# Autodesk Inventor assembly: Assembly1
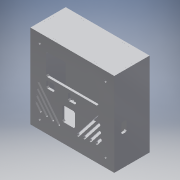
[picture p0: Inventor's stored thumbnail of the model, 180x180]
Saved by Autodesk Inventor 2018.2 (Build 222227000, 227)
## iProperties
Created: 2018-04-05
Part Number: Assembly1
Document SubType Name: Assembly
Designer: Derek
Author: Derek
## Documents named in this file (6)
- C:\Users\Derek Fronek\OneDrive\Documents\Digital Electronics\Finger Print Scanner\Case\Assembly1.iam
- C:\Users\Derek Fronek\OneDrive\Documents\Digital Electronics\Finger Print Scanner\Case\Side.ipt
- C:\Users\Derek Fronek\OneDrive\Documents\Digital Electronics\Finger Print Scanner\Case\Face.ipt
- C:\Users\Derek Fronek\OneDrive\Documents\Digital Electronics\Finger Print Scanner\Case\Side 2.ipt
- C:\Users\Derek Fronek\OneDrive\Documents\Digital Electronics\Finger Print Scanner\Case\top.ipt
- C:\Users\Derek Fronek\OneDrive\Documents\Digital Electronics\Finger Print Scanner\Case\Back.ipt
## Components (6 placed, 5 different names)
1. Face:1 — Flush:7, Flush:8, Flush:9, Mate:1, Flush:11
2. Side:2 — Flush:7, Flush:12
3. Side 2:1 — Flush:8
4. top:1 — Flush:9, Flush:10
5. Back:1 — Flush:10
6. top:2 — Mate:1, Flush:11, Flush:12
## Relationships (7: Flush 6, Mate 1)
- Flush:7: Face:1 ↔ Side:2
- Flush:8: Face:1 ↔ Side 2:1
- Flush:9: Face:1 ↔ top:1
- Flush:10: top:1 ↔ Back:1
- Mate:1: Face:1 ↔ top:2
- Flush:11: Face:1 ↔ top:2
- Flush:12: Side:2 ↔ top:2
